# Autodesk Inventor assembly: fullPCIconnector
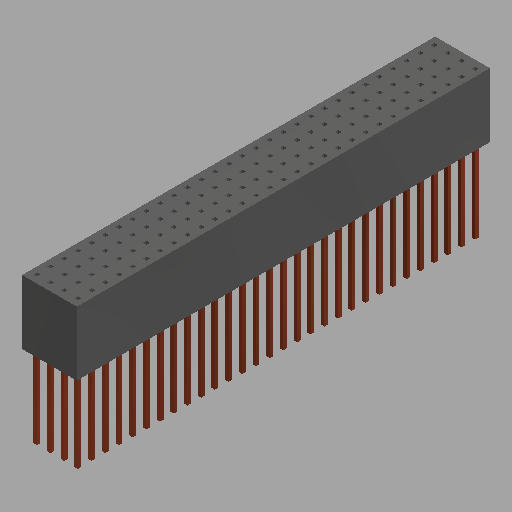
[picture p0: Inventor's stored thumbnail of the model, 512x512]
Saved by Autodesk Inventor 2022 (Build 260153000, 153)
## iProperties
Created: 2021-10-06
Part Number: fullPCIconnector
Document SubType Name: Assembly
Designer: Bowen O'Steen
Author: Bowen O'Steen
## Documents named in this file (3)
- C:\Users\gwhen\OneDrive\Desktop\Vault\Designs\MEMESat\MemeSat\Engineering Data\MemeSat\Subsystems\fullPCIconnector.iam
- C:\Users\gwhen\OneDrive\Desktop\Vault\Designs\MEMESat\MemeSat\Engineering Data\MemeSat\Subsystems\PCIconnector.ipt
- C:\Users\gwhen\OneDrive\Desktop\Vault\Designs\MEMESat\MemeSat\Engineering Data\MemeSat\Subsystems\PCIpins.ipt
## Components (2 placed, 2 different names)
1. PCIconnector:1 — Mate:1, Mate:2, Flush:1, Mate:3, Mate:4, Mate:5
2. PCIpins:1 — Mate:3, Mate:4, Mate:5
## Relationships (6: Mate 5, Flush 1)
- Mate:1: PCIconnector:1
- Mate:2: PCIconnector:1
- Flush:1: PCIconnector:1
- Mate:3: PCIconnector:1 ↔ PCIpins:1
- Mate:4: PCIconnector:1 ↔ PCIpins:1
- Mate:5 (-4.59 mm): PCIconnector:1 ↔ PCIpins:1
